# Autodesk Inventor assembly: ServoBlock
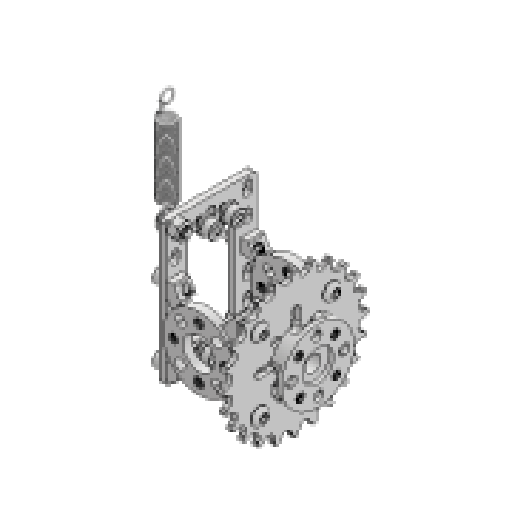
[picture p0: Inventor's stored thumbnail of the model, 512x512]
Saved by Autodesk Inventor 2023 (Build 270158000, 158)
## iProperties
Created: 2022-09-10
Part Number: ServoBlock
Document SubType Name: Assembly
Designer: deli
Author: deli
## Documents named in this file (6)
- C:\Users\deli\OneDrive - Eastside Preparatory School\FTC\8103-power-play\CAD\ServoBlock.iam
- C:\Users\deli\OneDrive - Eastside Preparatory School\FTC\8103-power-play\CAD\3311-0014-0024 with 19mm hole.ipt
- C:\Users\deli\OneDrive - Eastside Preparatory School\FTC\8103-power-play\CAD\FTC-parts\goBILDA\2802-0004-0010.ipt
- C:\Users\deli\OneDrive - Eastside Preparatory School\FTC\8103-power-play\CAD\FTC-parts\goBILDA\2812-0004-0007.ipt
- C:\Users\deli\OneDrive - Eastside Preparatory School\FTC\8103-power-play\CAD\FTC-parts\goBILDA\1221-0032-0001.ipt
- C:\Users\deli\OneDrive - Eastside Preparatory School\FTC\8103-power-play\CAD\FTC-parts\goBILDA\1603-0032-0008 assembly.ipt
## Components (10 placed, 5 different names)
1. 3311-0014-0024 with 19mm hole:1 — Mate:11, Mate:12, Mate:13, Mate:14, Mate:15, Mate:16
2. 2802-0004-0010:1 — Mate:12
3. 2802-0004-0010:2 — Mate:15, Mate:16
4. 2802-0004-0010:3 — Mate:11, Mate:13
5. 2802-0004-0010:4 — Mate:14
6. 2812-0004-0007:1
7. 1221-0032-0001:1 — Mate:17, Mate:18, Mate:19, Mate:20, Mate:21, Mate:22
8. 1603-0032-0008 assembly:1 — Mate:19, Mate:20, Mate:21, Mate:23, Mate:24
9. 1603-0032-0008 assembly:2 — Mate:17, Mate:18, Mate:22
10. 1221-0032-0001:2 — Mate:23, Mate:24
## Relationships (16: Mate 16)
- [Mate]: 3311-0014-0024 with 19mm hole:1 ↔ 2802-0004-0010:4
- [Mate]: 3311-0014-0024 with 19mm hole:1 ↔ 2802-0004-0010:1
- Mate:11: 3311-0014-0024 with 19mm hole:1 ↔ 2802-0004-0010:3
- Mate:12: 3311-0014-0024 with 19mm hole:1 ↔ 2802-0004-0010:1
- Mate:13: 3311-0014-0024 with 19mm hole:1 ↔ 2802-0004-0010:3
- Mate:14: 3311-0014-0024 with 19mm hole:1 ↔ 2802-0004-0010:4
- Mate:15: 3311-0014-0024 with 19mm hole:1 ↔ 2802-0004-0010:2
- Mate:16: 3311-0014-0024 with 19mm hole:1 ↔ 2802-0004-0010:2
- Mate:17: 1221-0032-0001:1 ↔ 1603-0032-0008 assembly:2
- Mate:18: 1221-0032-0001:1 ↔ 1603-0032-0008 assembly:2
- Mate:19: 1221-0032-0001:1 ↔ 1603-0032-0008 assembly:1
- Mate:20: 1221-0032-0001:1 ↔ 1603-0032-0008 assembly:1
- Mate:21: 1221-0032-0001:1 ↔ 1603-0032-0008 assembly:1
- Mate:22: 1221-0032-0001:1 ↔ 1603-0032-0008 assembly:2
- Mate:23: 1603-0032-0008 assembly:1 ↔ 1221-0032-0001:2
- Mate:24: 1603-0032-0008 assembly:1 ↔ 1221-0032-0001:2
